# Autodesk Inventor assembly: assembly
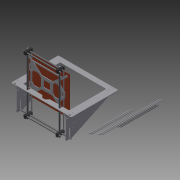
[picture p0: Inventor's stored thumbnail of the model, 180x180]
Saved by Autodesk Inventor 2013 (Build 170138000, 138)
## iProperties
Created: 2013-11-17
Part Number: assembly
Document SubType Name: Assembly
Designer: Masta
Author: Masta
## Documents named in this file (13)
- D:\prusa i3\assembly\assembly.iam
- D:\prusa i3\assembly\lasercut_aluminium\caddy.ipt
- D:\prusa i3\assembly\lasercut_aluminium\main_frame.ipt
- D:\prusa i3\assembly\lasercut_aluminium\side_frame.ipt
- D:\prusa i3\assembly\other\fi8x320.ipt
- D:\prusa i3\assembly\other\fi8x450.ipt
- D:\prusa i3\assembly\other\fi8x470.ipt
- D:\prusa i3\assembly\other\M5x300.ipt
- D:\prusa i3\assembly\other\M10x480.ipt
- D:\prusa i3\assembly\other\haetbed300.ipt
- D:\prusa i3\assembly\plastics\Y_corner.ipt
- D:\prusa i3\assembly\other\M10x290.ipt
- D:\prusa i3\assembly\other\M10x410.ipt
## Components (23 placed, 12 different names)
1. main_frame:1 — Mate:1, Flush:3, Mate:2, Mate:3, Mate:4, Flush:4, Insert:1, Insert:2
2. caddy:1 — Mate:4, Flush:4, Insert:4, Insert:5
3. side_frame:1 — Flush:1, Flush:2, Flush:3, Mate:3, Flush:9
4. side_frame:2 — Flush:1, Mate:1, Flush:2, Mate:2
5. fi8x320:1
6. fi8x320:2
7. fi8x450:1 — Tangent:18, Tangent:19, Mate:7, Mate:8
8. fi8x450:2 — Tangent:16, Tangent:17, Mate:5, Mate:6
9. fi8x470:1
10. fi8x470:2
11. M5x300:1
12. M5x300:2
13. M10x480:1 — Insert:1, Tangent:10, Tangent:11, Tangent:12, Tangent:13, Flush:7
14. M10x480:2 — Insert:2, Tangent:8, Tangent:9, Tangent:14, Tangent:15
15. haetbed300:1 — Insert:4, Insert:5
16. Y_corner:1 — Tangent:6, Angle:2, Tangent:12, Tangent:13, Tangent:18, Tangent:19, Mate:7, Flush:6, Flush:7
17. Y_corner:2 — Tangent:5, Flush:5, Tangent:7, Angle:1, Tangent:14, Tangent:15, Tangent:16, Tangent:17, Mate:5, Flush:6, Tangent:20, Tangent:21
18. Y_corner:3 — Angle:4, Tangent:10, Tangent:11, Mate:8
19. Y_corner:4 — Angle:3, Tangent:8, Tangent:9, Mate:6, Tangent:22, Tangent:23, Tangent:24, Tangent:25
20. M10x290:1 — Tangent:5, Tangent:6, Flush:5, Tangent:7, Flush:8
21. M10x290:2 — Tangent:24, Tangent:25, Flush:10
22. M10x290:3 — Tangent:20, Tangent:21, Flush:8, Flush:10
23. M10x410:1 — Tangent:22, Tangent:23, Flush:9
## Relationships (47: Tangent 21, Flush 10, Mate 8, Insert 4, Angle 4)
- Flush:1: side_frame:1 ↔ side_frame:2
- Mate:1: main_frame:1 ↔ side_frame:2
- Flush:2: side_frame:1 ↔ side_frame:2
- Flush:3: main_frame:1 ↔ side_frame:1
- Mate:2 (0.25 mm): main_frame:1 ↔ side_frame:2
- Mate:3 (0.25 mm): main_frame:1 ↔ side_frame:1
- Mate:4 (5 mm): main_frame:1 ↔ caddy:1
- Flush:4: main_frame:1 ↔ caddy:1
- Insert:1 (-200 mm): main_frame:1 ↔ M10x480:1
- Insert:2 (-200 mm): main_frame:1 ↔ M10x480:2
- Insert:4 (10 mm): caddy:1 ↔ haetbed300:1
- Insert:5 (10 mm): caddy:1 ↔ haetbed300:1
- Tangent:5: Y_corner:2 ↔ M10x290:1
- Tangent:6: Y_corner:1 ↔ M10x290:1
- Flush:5 (-11 mm): Y_corner:2 ↔ M10x290:1
- Tangent:7: Y_corner:2 ↔ M10x290:1
- Angle:1 (0 deg): Y_corner:2
- Angle:2 (0 deg): Y_corner:1
- Angle:3 (180 deg): Y_corner:4
- Angle:4 (0 deg): Y_corner:3
- Tangent:8: M10x480:2 ↔ Y_corner:4
- Tangent:9: M10x480:2 ↔ Y_corner:4
- Tangent:10: M10x480:1 ↔ Y_corner:3
- Tangent:11: M10x480:1 ↔ Y_corner:3
- Tangent:12: M10x480:1 ↔ Y_corner:1
- Tangent:13: M10x480:1 ↔ Y_corner:1
- Tangent:14: M10x480:2 ↔ Y_corner:2
- Tangent:15: M10x480:2 ↔ Y_corner:2
- Tangent:16: fi8x450:2 ↔ Y_corner:2
- Tangent:17: fi8x450:2 ↔ Y_corner:2
- Mate:5: fi8x450:2 ↔ Y_corner:2
- Mate:6: fi8x450:2 ↔ Y_corner:4
- Tangent:18: fi8x450:1 ↔ Y_corner:1
- Tangent:19: fi8x450:1 ↔ Y_corner:1
- Mate:7: fi8x450:1 ↔ Y_corner:1
- Mate:8: fi8x450:1 ↔ Y_corner:3
- Flush:6: Y_corner:1 ↔ Y_corner:2
- Flush:7 (13 mm): M10x480:1 ↔ Y_corner:1
- Tangent:20: Y_corner:2 ↔ M10x290:3
- Tangent:21: Y_corner:2 ↔ M10x290:3
- Flush:8: M10x290:1 ↔ M10x290:3
- Tangent:22: Y_corner:4 ↔ M10x410:1
- Tangent:23: Y_corner:4 ↔ M10x410:1
- Flush:9 (-11 mm): side_frame:1 ↔ M10x410:1
- Tangent:24: Y_corner:4 ↔ M10x290:2
- Tangent:25: Y_corner:4 ↔ M10x290:2
- Flush:10: M10x290:2 ↔ M10x290:3
